# Autodesk Inventor assembly: RAI_Assembly
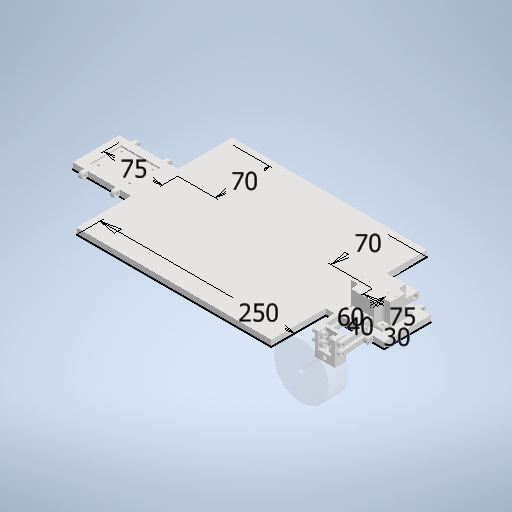
[picture p0: Inventor's stored thumbnail of the model, 512x512]
Saved by Autodesk Inventor 2025.2 (Build 292293000, 293)
## iProperties
Created: 2025-01-03
Part Number: RAI_Assembly
Document SubType Name: Assembly
Designer: SEON
Author: SEON
## Documents named in this file (7)
- C:\Users\SEON\Documents\Inventor\ProjectRAI\RAI_Assembly.iam
- C:\Users\SEON\Documents\Inventor\ProjectRAI\BottomFrame.ipt
- C:\Users\SEON\Documents\Inventor\ProjectRAI\SuspensionSupporter.ipt
- C:\Users\SEON\Documents\Inventor\ProjectRAI\TireDummy.ipt
- C:\Users\SEON\Documents\Inventor\ProjectRAI\SteeringFrame.ipt
- C:\Users\SEON\Documents\Inventor\ProjectRAI\SteeringConnector.ipt
- C:\Users\SEON\Documents\Inventor\ProjectRAI\SuspensionFrame.ipt
## Components (13 placed, 6 different names)
1. BottomFrame:1 — 메이트:1, 메이트:2, 메이트:3, 메이트:5, 메이트:6, 메이트:17, 메이트:18, 메이트:21
2. SuspensionSupporter:1 — 메이트:1, 메이트:2, 메이트:3, 메이트:4
3. SuspensionSupporter:2 — 메이트:4, 메이트:5, 메이트:6, 메이트:23, 메이트:26
4. TireDummy:1 — 메이트:7, 메이트:8
5. SteeringFrame:1 — 메이트:7, 메이트:8, 메이트:9, 메이트:10, 메이트:11, 메이트:12, 메이트:19, 메이트:24, 메이트:27, 메이트:28, 메이트:29, 메이트:30
6. SuspensionFrame:2 — 메이트:13, 메이트:14, 메이트:18, 메이트:21
7. SteeringConnector:3 — 메이트:9, 메이트:10, 메이트:13, 메이트:14
8. SteeringConnector:4 — 메이트:11, 메이트:12, 메이트:15, 메이트:16
9. SuspensionFrame:3 — 메이트:15, 메이트:16, 메이트:17
10. SuspensionFrame:4 — 메이트:19, 메이트:23, 메이트:31
11. SuspensionFrame:5 — 메이트:24, 메이트:26, 메이트:32
12. SteeringConnector:5 — 메이트:27, 메이트:28, 메이트:32
13. SteeringConnector:6 — 메이트:29, 메이트:30, 메이트:31
## Relationships (29: Mate 29)
- 메이트:1 [Mate]: BottomFrame:1 ↔ SuspensionSupporter:1
- 메이트:2 [Mate]: BottomFrame:1 ↔ SuspensionSupporter:1
- 메이트:3 [Mate]: BottomFrame:1 ↔ SuspensionSupporter:1
- 메이트:4 [Mate]: SuspensionSupporter:1 ↔ SuspensionSupporter:2
- 메이트:5 [Mate]: BottomFrame:1 ↔ SuspensionSupporter:2
- 메이트:6 [Mate]: BottomFrame:1 ↔ SuspensionSupporter:2
- 메이트:7 [Mate]: TireDummy:1 ↔ SteeringFrame:1
- 메이트:8 [Mate] (5 mm): TireDummy:1 ↔ SteeringFrame:1
- 메이트:9 [Mate]: SteeringFrame:1 ↔ SteeringConnector:3
- 메이트:10 [Mate]: SteeringFrame:1 ↔ SteeringConnector:3
- 메이트:11 [Mate]: SteeringFrame:1 ↔ SteeringConnector:4
- 메이트:12 [Mate]: SteeringFrame:1 ↔ SteeringConnector:4
- 메이트:13 [Mate]: SuspensionFrame:2 ↔ SteeringConnector:3
- 메이트:14 [Mate]: SuspensionFrame:2 ↔ SteeringConnector:3
- 메이트:15 [Mate]: SteeringConnector:4 ↔ SuspensionFrame:3
- 메이트:16 [Mate]: SteeringConnector:4 ↔ SuspensionFrame:3
- 메이트:17 [Mate]: BottomFrame:1 ↔ SuspensionFrame:3
- 메이트:18 [Mate]: BottomFrame:1 ↔ SuspensionFrame:2
- 메이트:19 [Mate]: SteeringFrame:1 ↔ SuspensionFrame:4
- 메이트:21 [Mate]: BottomFrame:1 ↔ SuspensionFrame:2
- 메이트:23 [Mate]: SuspensionSupporter:2 ↔ SuspensionFrame:4
- 메이트:24 [Mate]: SteeringFrame:1 ↔ SuspensionFrame:5
- 메이트:26 [Mate]: SuspensionSupporter:2 ↔ SuspensionFrame:5
- 메이트:27 [Mate]: SteeringFrame:1 ↔ SteeringConnector:5
- 메이트:28 [Mate]: SteeringFrame:1 ↔ SteeringConnector:5
- 메이트:29 [Mate]: SteeringFrame:1 ↔ SteeringConnector:6
- 메이트:30 [Mate]: SteeringFrame:1 ↔ SteeringConnector:6
- 메이트:31 [Mate]: SuspensionFrame:4 ↔ SteeringConnector:6
- 메이트:32 [Mate]: SuspensionFrame:5 ↔ SteeringConnector:5
